# Autodesk Inventor assembly: Helix DLP V2
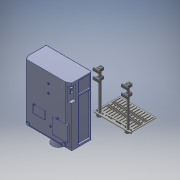
[picture p0: Inventor's stored thumbnail of the model, 180x180]
Saved by Autodesk Inventor 2019 (Build 230136000, 136)
## iProperties
Created: 2020-11-30
Part Number: Helix DLP V2
Document SubType Name: Assembly
Designer: Vijay
Author: Vijay
## Documents named in this file (7)
- C:\Users\Vijay\Documents\GitHub\Helix-DLP-3D-Printer\Helix DLP V2\Helix DLP V2.iam
- C:\Users\Vijay\Documents\GitHub\Helix-DLP-3D-Printer\Helix DLP V2\OTS Componenets\Projector.ipt
- C:\Users\Vijay\Documents\GitHub\Helix-DLP-3D-Printer\Helix DLP V2\Build Plate.ipt
- C:\Users\Vijay\Documents\GitHub\Helix-DLP-3D-Printer\Helix DLP V2\Z Shaft.ipt
- C:\Users\Vijay\Documents\GitHub\Helix-DLP-3D-Printer\Helix DLP V2\OTS Componenets\108110252-9-support_shf16\support_shf16.ipt
- C:\Users\Vijay\Documents\Inventor\Content Center Files\R2019\en-US\AS 1420\AS 1420 - 1973 - M5 x 20.ipt
- C:\Users\Vijay\Documents\GitHub\Helix-DLP-3D-Printer\Helix DLP V2\OTS Componenets\108111903-9-support_sk16\support_sk16.ipt
## Components (14 placed, 6 different names)
1. Projector:1
2. Build Plate:1 — Mate:3, Flush:4, Flush:5, Flush:6, Flush:7, Insert:1, Insert:2, Insert:3, Insert:4
3. Z Shaft:1 — Mate:1, Flush:1, Mate:4, Mate:7, Flush:11
4. Z Shaft:2 — Mate:2, Flush:2, Mate:5, Mate:6, Flush:12
5. support_shf16:1 — Mate:1, Flush:1, Flush:3, Mate:3, Flush:4, Flush:6
6. support_shf16:2 — Mate:2, Flush:2, Flush:3, Flush:5, Flush:7
7. AS 1420 - Metric M5 x 20:1 — Insert:1
8. AS 1420 - Metric M5 x 20:2 — Insert:2
9. AS 1420 - Metric M5 x 20:3 — Insert:3
10. AS 1420 - Metric M5 x 20:4 — Insert:4
11. support_sk16:1 — Mate:4, Flush:8, Flush:11
12. support_sk16:2 — Mate:5, Flush:9, Flush:12, Mate:8
13. support_sk16:3 — Mate:6, Flush:9, Flush:10, Flush:13, Mate:8
14. support_sk16:4 — Mate:7, Flush:8, Flush:10, Flush:13
## Relationships (25: Flush 13, Mate 8, Insert 4)
- Mate:1: Z Shaft:1 ↔ support_shf16:1
- Mate:2: Z Shaft:2 ↔ support_shf16:2
- Flush:1: Z Shaft:1 ↔ support_shf16:1
- Flush:2: Z Shaft:2 ↔ support_shf16:2
- Flush:3: support_shf16:1 ↔ support_shf16:2
- Mate:3: Build Plate:1 ↔ support_shf16:1
- Flush:4: Build Plate:1 ↔ support_shf16:1
- Flush:5: Build Plate:1 ↔ support_shf16:2
- Flush:6 (5 mm): Build Plate:1 ↔ support_shf16:1
- Flush:7 (5 mm): Build Plate:1 ↔ support_shf16:2
- Insert:1: Build Plate:1 ↔ AS 1420 - Metric M5 x 20:1
- Insert:2: Build Plate:1 ↔ AS 1420 - Metric M5 x 20:2
- Insert:3: Build Plate:1 ↔ AS 1420 - Metric M5 x 20:3
- Insert:4: Build Plate:1 ↔ AS 1420 - Metric M5 x 20:4
- Mate:4: Z Shaft:1 ↔ support_sk16:1
- Mate:5: Z Shaft:2 ↔ support_sk16:2
- Mate:6: Z Shaft:2 ↔ support_sk16:3
- Mate:7: Z Shaft:1 ↔ support_sk16:4
- Flush:8: support_sk16:1 ↔ support_sk16:4
- Flush:9: support_sk16:2 ↔ support_sk16:3
- Flush:10: support_sk16:3 ↔ support_sk16:4
- Flush:11: Z Shaft:1 ↔ support_sk16:1
- Flush:12: Z Shaft:2 ↔ support_sk16:2
- Flush:13: support_sk16:3 ↔ support_sk16:4
- Mate:8 (40 mm): support_sk16:2 ↔ support_sk16:3
